# Autodesk Inventor assembly: Side Plate Assembly_MIR
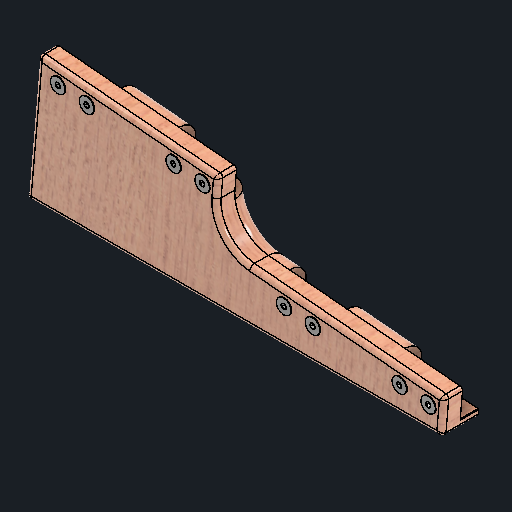
[picture p0: Inventor's stored thumbnail of the model, 512x512]
Saved by Autodesk Inventor 2026.2 (Build 302298000, 298)
## iProperties
Created: 2026-10-06
Part Number: Side Plate Assembly_MIR
Document SubType Name: Assembly
Designer: Joshua Eah
Author: Joshua Eah
## Documents named in this file (3)
- C:\Users\Joshua Eah\Documents\GitHub\designs\Guitar\Modular Pedalboard\Side Plate Assembly_MIR.iam
- C:\Users\Joshua Eah\Documents\GitHub\designs\Guitar\Modular Pedalboard\Side_MIR.ipt
- C:\Users\Joshua Eah\Documents\GitHub\designs\Guitar\Modular Pedalboard\Hardware\Fasteners\M5x0.8x20mm FHCS.ipt
## Components (9 placed, 2 different names)
1. Side_MIR:1 — Insert:1
2. M5x0.8x20mm FHCS:1 — Insert:1
3. M5x0.8x20mm FHCS:2
4. M5x0.8x20mm FHCS:3
5. M5x0.8x20mm FHCS:4
6. M5x0.8x20mm FHCS:5
7. M5x0.8x20mm FHCS:6
8. M5x0.8x20mm FHCS:7
9. M5x0.8x20mm FHCS:8
## Relationships (1: Insert 1)
- Insert:1: Side_MIR:1 ↔ M5x0.8x20mm FHCS:1
